# Autodesk Inventor assembly: stackapproximateassembly
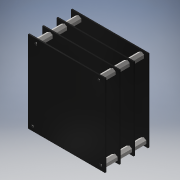
[picture p0: Inventor's stored thumbnail of the model, 180x180]
Saved by Autodesk Inventor 2022 (Build 260153000, 153)
## iProperties
Created: 2021-04-30
Part Number: stackapproximateassembly
Document SubType Name: Assembly
Designer: Bowen O'Steen
Author: Bowen O'Steen
## Documents named in this file (3)
- C:\$WorkingFolder\Engineering Data\MemeSat\Assembly\stackapproximateassembly.iam
- C:\$WorkingFolder\Engineering Data\MemeSat\Internal Components\pc104standard.ipt
- C:\$WorkingFolder\Engineering Data\MemeSat\Internal Components\pc104standoff.ipt
## Components (16 placed, 2 different names)
1. pc104standard:1 — Mate:1, Mate:2, Mate:3, Mate:4, Mate:5, Mate:6, Mate:7, Mate:8, Flush:1, Mate:9, Mate:10, Mate:11, Mate:12, Mate:13, Mate:14, Mate:15, Mate:16, Angle:1, Angle:2, Angle:3, Angle:4
2. pc104standard:2 — Mate:1, Mate:2, Mate:17, Mate:18, Mate:19, Mate:20, Mate:21, Mate:22, Mate:23, Mate:24, Mate:25, Angle:5, Angle:6, Angle:7, Angle:8
3. pc104standard:3 — Mate:3, Mate:4, Mate:26, Mate:27, Mate:28, Mate:29, Mate:30, Mate:31, Mate:32, Mate:33, Mate:34, Angle:9, Angle:10, Angle:11, Angle:12
4. pc104standard:4 — Mate:5, Mate:6, Mate:35
5. pc104standoff:1 — Mate:10, Mate:14, Angle:3
6. pc104standoff:2 — Mate:12, Mate:13, Angle:4
7. pc104standoff:3 — Mate:11, Mate:16, Angle:2
8. pc104standoff:4 — Mate:9, Mate:15, Mate:17, Angle:1
9. pc104standoff:5 — Mate:18, Mate:23, Angle:5
10. pc104standoff:6 — Mate:19, Mate:22, Angle:8
11. pc104standoff:7 — Mate:21, Mate:25, Mate:26, Angle:7
12. pc104standoff:8 — Mate:20, Mate:24, Angle:6
13. pc104standoff:9 — Mate:27, Mate:32, Angle:11
14. pc104standoff:10 — Mate:29, Mate:34, Mate:35, Angle:9
15. pc104standoff:11 — Mate:28, Mate:33, Angle:12
16. pc104standoff:12 — Mate:30, Mate:31, Angle:10
## Relationships (48: Mate 35, Angle 12, Flush 1)
- Mate:1: pc104standard:1 ↔ pc104standard:2
- Mate:2: pc104standard:1 ↔ pc104standard:2
- Mate:3: pc104standard:1 ↔ pc104standard:3
- Mate:4: pc104standard:1 ↔ pc104standard:3
- Mate:5: pc104standard:1 ↔ pc104standard:4
- Mate:6: pc104standard:1 ↔ pc104standard:4
- Mate:7: pc104standard:1
- Mate:8: pc104standard:1
- Flush:1: pc104standard:1
- Mate:9: pc104standard:1 ↔ pc104standoff:4
- Mate:10: pc104standard:1 ↔ pc104standoff:1
- Mate:11: pc104standard:1 ↔ pc104standoff:3
- Mate:12: pc104standard:1 ↔ pc104standoff:2
- Mate:13: pc104standard:1 ↔ pc104standoff:2
- Mate:14: pc104standard:1 ↔ pc104standoff:1
- Mate:15: pc104standard:1 ↔ pc104standoff:4
- Mate:16: pc104standard:1 ↔ pc104standoff:3
- Mate:17: pc104standard:2 ↔ pc104standoff:4
- Mate:18: pc104standard:2 ↔ pc104standoff:5
- Mate:19: pc104standard:2 ↔ pc104standoff:6
- Mate:20: pc104standard:2 ↔ pc104standoff:8
- Mate:21: pc104standard:2 ↔ pc104standoff:7
- Mate:22: pc104standard:2 ↔ pc104standoff:6
- Mate:23: pc104standard:2 ↔ pc104standoff:5
- Mate:24: pc104standard:2 ↔ pc104standoff:8
- Mate:25: pc104standard:2 ↔ pc104standoff:7
- Mate:26: pc104standard:3 ↔ pc104standoff:7
- Mate:27: pc104standard:3 ↔ pc104standoff:9
- Mate:28: pc104standard:3 ↔ pc104standoff:11
- Mate:29: pc104standard:3 ↔ pc104standoff:10
- Mate:30: pc104standard:3 ↔ pc104standoff:12
- Mate:31: pc104standard:3 ↔ pc104standoff:12
- Mate:32: pc104standard:3 ↔ pc104standoff:9
- Mate:33: pc104standard:3 ↔ pc104standoff:11
- Mate:34: pc104standard:3 ↔ pc104standoff:10
- Mate:35: pc104standard:4 ↔ pc104standoff:10
- Angle:1 (0 deg): pc104standard:1 ↔ pc104standoff:4
- Angle:2 (0 deg): pc104standard:1 ↔ pc104standoff:3
- Angle:3 (0 deg): pc104standard:1 ↔ pc104standoff:1
- Angle:4 (0 deg): pc104standard:1 ↔ pc104standoff:2
- Angle:5 (0 deg): pc104standard:2 ↔ pc104standoff:5
- Angle:6 (0 deg): pc104standard:2 ↔ pc104standoff:8
- Angle:7 (0 deg): pc104standard:2 ↔ pc104standoff:7
- Angle:8 (0 deg): pc104standard:2 ↔ pc104standoff:6
- Angle:9 (0 deg): pc104standard:3 ↔ pc104standoff:10
- Angle:10 (0 deg): pc104standard:3 ↔ pc104standoff:12
- Angle:11 (0 deg): pc104standard:3 ↔ pc104standoff:9
- Angle:12 (0 deg): pc104standard:3 ↔ pc104standoff:11
